# Autodesk Inventor assembly: Assembly2
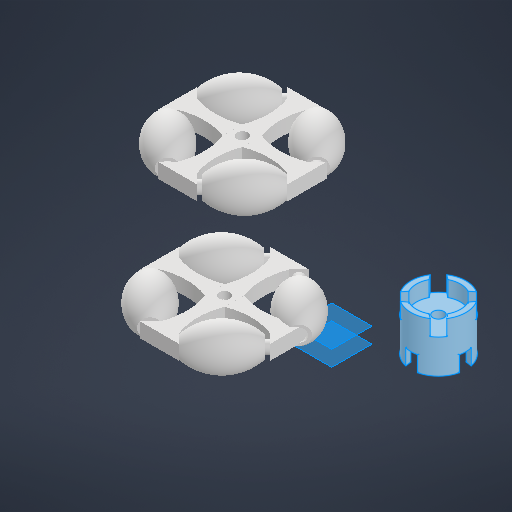
[picture p0: Inventor's stored thumbnail of the model, 512x512]
Saved by Autodesk Inventor 2026 (Build 300175000, 175)
## iProperties
Created: 2025-10-16
Part Number: Assembly2
Document SubType Name: Assembly
Designer: masak
Author: masak
## Documents named in this file (5)
- C:\Robohan\CAD\オムニ\Assembly2.iam
- C:\Robohan\CAD\オムニ\フレームD.ipt
- C:\Robohan\CAD\オムニ\フレームL.ipt
- C:\Robohan\CAD\オムニ\ホイール.ipt
- C:\Robohan\CAD\オムニ\隙間パーツ.ipt
## Components (13 placed, 4 different names)
1. フレームD:1 — 挿入:2, メイト:3, メイト:4, メイト:6
2. フレームL:1 — 挿入:1, 挿入:2, メイト:3, メイト:5
3. ホイール:1 — 挿入:1
4. ホイール:3 — メイト:4
5. ホイール:4 — メイト:5
6. ホイール:5 — メイト:6
7. フレームD:2
8. フレームL:2
9. ホイール:6
10. ホイール:7
11. ホイール:8
12. ホイール:9
13. 隙間パーツ:1
## Relationships (12: Mate 8, Insert 4)
- 挿入:1 [Insert] (0.5 mm): フレームL:1 ↔ ホイール:1
- 挿入:2 [Insert]: フレームD:1 ↔ フレームL:1
- メイト:3 [Mate]: フレームD:1 ↔ フレームL:1
- メイト:4 [Mate]: フレームD:1 ↔ ホイール:3
- メイト:5 [Mate]: フレームL:1 ↔ ホイール:4
- メイト:6 [Mate]: フレームD:1 ↔ ホイール:5
- [Insert] (0.5 mm): フレームL:2 ↔ ホイール:6
- [Insert]: フレームD:2 ↔ フレームL:2
- [Mate]: フレームD:2 ↔ フレームL:2
- [Mate]: フレームD:2 ↔ ホイール:7
- [Mate]: フレームL:2 ↔ ホイール:8
- [Mate]: フレームD:2 ↔ ホイール:9
## Named parameters: d8_d2 = 0.5 mm, d9_d3 = 0 mm, d10_d4 = 0 mm, d11_d5 = 0 mm, d12_d6 = 0 mm, d13_d7 = 0 mm
